# Autodesk Inventor assembly: main
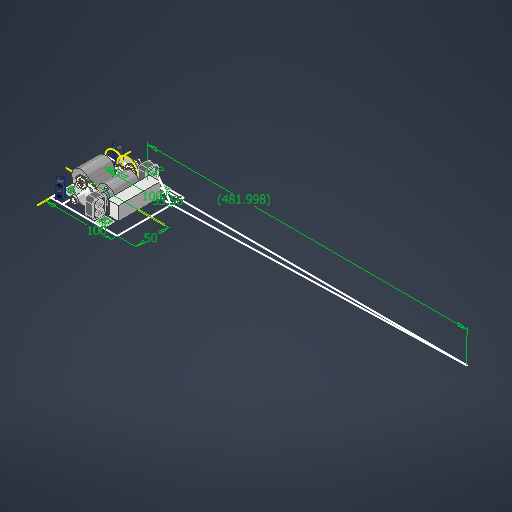
[picture p0: Inventor's stored thumbnail of the model, 512x512]
Saved by Autodesk Inventor 2026.2 (Build 302298000, 298)
## iProperties
Created: 2026-03-09
Part Number: main
Document SubType Name: Assembly
Designer: szymo
Author: szymo
## Documents named in this file (6)
- C:\Users\szymo\Downloads\evangelion-turbo\inventor-project\main.iam
- C:\Users\szymo\Downloads\evangelion-turbo\inventor-project\drive-train.iam
- C:\Users\szymo\Downloads\evangelion-turbo\inventor-project\LUNA.ipt
- C:\Users\szymo\Downloads\evangelion-turbo\inventor-project\3s450mah.ipt
- C:\Users\szymo\Downloads\evangelion-turbo\inventor-project\sharp\sharp\sharp.ipt
- C:\Users\szymo\Downloads\evangelion-turbo\inventor-project\KTIR-Board.ipt
## Components (10 placed, 5 different names)
1. drive-train:1 [sub-assembly] — Flush:2, Flush:3, Flush:4, Mate:2, Mate:3, Tangent:1
2. 3s450mah:1 — Flush:8, Tangent:1, Flush:9
3. KTIR-Board:3 — Flush:18, Flush:20, Mate:9
4. KTIR-Board:4 — Flush:17, Flush:19, Flush:21
5. sharp:2 — Angle:3, Flush:15, Mate:6, Mate:8
6. sharp:3 — Angle:4, Flush:16, Mate:5, Mate:7
7. LUNA:2 — Mate:1, Mate:3, Angle:2, Flush:7
8. LUNA:1 — Flush:5, Mate:2, Angle:1, Flush:6
9. KTIR-Board:1 — Flush:10, Flush:11, Flush:13
10. KTIR-Board:2 — Mate:4, Flush:12, Flush:14
## Relationships (35: Flush 21, Mate 9, Angle 4, Tangent 1)
- Flush:1 (-101.75 mm)
- Flush:2: drive-train:1
- Flush:3 (-18.4 mm): drive-train:1
- Flush:4: drive-train:1
- Flush:5 (49.5 mm): LUNA:1
- Mate:1 (-49.5 mm): LUNA:2
- Mate:2 (18 mm): drive-train:1 ↔ LUNA:1
- Mate:3 (18 mm): drive-train:1 ↔ LUNA:2
- Angle:1 (0 deg): LUNA:1
- Angle:2 (180 deg): LUNA:2
- Flush:6: LUNA:1
- Flush:7: LUNA:2
- Flush:8 (1 mm): 3s450mah:1
- Tangent:1: drive-train:1 ↔ 3s450mah:1
- Flush:9 (-31 mm): 3s450mah:1
- Flush:10 (-49.5 mm): KTIR-Board:1
- Mate:4 (-49.5 mm): KTIR-Board:2
- Flush:11 (0.13 mm): KTIR-Board:1
- Flush:12 (0.13 mm): KTIR-Board:2
- Flush:13 (67 mm): KTIR-Board:1
- Flush:14 (-67 mm): KTIR-Board:2
- Angle:3 (210 deg): sharp:2
- Angle:4 (-150 deg): sharp:3
- Flush:15 (0.5 mm): sharp:2
- Flush:16 (0.5 mm): sharp:3
- Mate:5 (-1 mm): sharp:3
- Mate:6 (-1 mm): sharp:2
- Mate:7 (-49.5 mm): sharp:3
- Mate:8 (49.5 mm): sharp:2
- Flush:17: KTIR-Board:4
- Flush:18: KTIR-Board:3
- Flush:19 (2 mm): KTIR-Board:4
- Flush:20 (2 mm): KTIR-Board:3
- Flush:21 (-21 mm): KTIR-Board:4
- Mate:9 (21 mm): KTIR-Board:3
